# Autodesk Inventor assembly: LowerBody
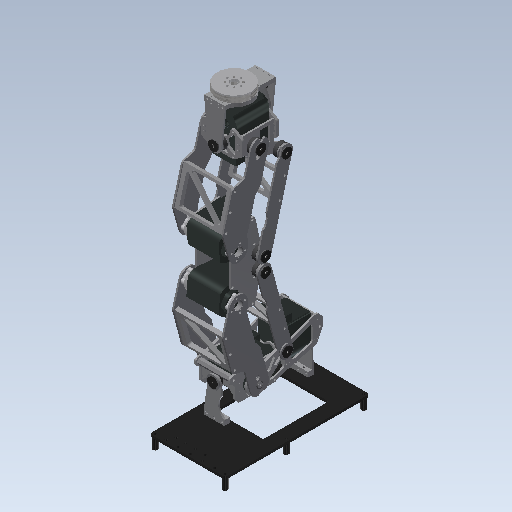
[picture p0: Inventor's stored thumbnail of the model, 512x512]
Saved by Autodesk Inventor 2020.4 (Build 244396000, 396)
## iProperties
Created: 2016-08-23
Part Number: LowerBody
Material: 一般
Document SubType Name: Assembly
Designer: hiro
Mass: 982.556 g
Surface Area: 2608.59 cm^2
Volume: 455.691 cm^3
Density: 2.15619 g/cm^3
Author: hiro
## Documents named in this file (12)
- C:\Users\Masato\Documents\Inventor\CIT Brains_Inventor\OpenPlatform_ver3_0\LowerBody.iam
- C:\Users\Masato\Documents\Inventor\CIT Brains_Inventor\OpenPlatform_ver3_0\下半身\足首\足首_1.iam
- C:\Users\Masato\Documents\Inventor\CIT Brains_Inventor\OpenPlatform_ver3_0\下半身\足首\足首_独立ピッチ_1.iam
- C:\Users\Masato\Documents\Inventor\CIT Brains_Inventor\OpenPlatform_ver3_0\下半身\リンク\LowerFrontLink.iam
- C:\Users\Masato\Documents\Inventor\CIT Brains_Inventor\OpenPlatform_ver3_0\下半身\付け根ロール\付け根ロール_1.iam
- C:\Users\Masato\Documents\Inventor\CIT Brains_Inventor\OpenPlatform_ver3_0\下半身\リンク\LowerBackLink.iam
- C:\Users\Masato\Documents\Inventor\CIT Brains_Inventor\OpenPlatform_ver3_0\下半身\長穴減速\長穴減速_ホーン.iam
- C:\Users\Masato\Documents\Inventor\CIT Brains_Inventor\OpenPlatform_ver3_0\下半身\膝\膝_1.iam
- C:\Users\Masato\Documents\Inventor\CIT Brains_Inventor\OpenPlatform_ver3_0\下半身\付け根\付け根_1.iam
- C:\Users\Masato\Documents\Inventor\CIT Brains_Inventor\OpenPlatform_ver3_0\下半身\リンク\UpperBackLink.iam
- C:\Users\Masato\Documents\Inventor\CIT Brains_Inventor\OpenPlatform_ver3_0\下半身\リンク\UpperFrontLink.iam
- C:\Users\Masato\Documents\Inventor\CIT Brains_Inventor\OpenPlatform_ver3_0\下半身\足裏\foot.iam
## Components (12 placed, 11 different names)
1. 付け根ロール_1:1 [sub-assembly] — メイト:23, フラッシュ:25, フラッシュ:26, 挿入:97, 角度:4, 角度:8, 角度:12, 挿入:123
2. 長穴減速_ホーン:1 [sub-assembly] — 挿入:97, 挿入:109
3. 付け根_1:1 [sub-assembly] — 角度:4, 挿入:109, 挿入:112, 挿入:113, 挿入:123
4. UpperFrontLink:1 [sub-assembly] — 挿入:111, 挿入:112, 角度:12
5. UpperBackLink:1 [sub-assembly] — 挿入:113, 挿入:114
6. 膝_1:1 [sub-assembly] — 挿入:98, 挿入:111, 挿入:114, 挿入:115
7. LowerFrontLink:2 [sub-assembly] — 挿入:98, 角度:11, 挿入:118
8. LowerBackLink:1 [sub-assembly] — 挿入:115, 挿入:120, 挿入:122
9. 足首_1:1 [sub-assembly] — 挿入:117, 挿入:119, 挿入:121
10. 足首_独立ピッチ_1:1 [sub-assembly] — 挿入:118, 挿入:119, 挿入:120
11. 足首_独立ピッチ_1:2 [sub-assembly] — 挿入:121, 挿入:122
12. Foot:1 [sub-assembly] — 角度:8, 挿入:117, 角度:11
## Relationships (22: Insert 15, Angle 4, Flush 2, Mate 1)
- メイト:23 [Mate]: 付け根ロール_1:1
- フラッシュ:25 [Flush]: 付け根ロール_1:1
- フラッシュ:26 [Flush]: 付け根ロール_1:1
- 挿入:97 [Insert]: 付け根ロール_1:1 ↔ 長穴減速_ホーン:1
- 挿入:98 [Insert]: 膝_1:1 ↔ LowerFrontLink:2
- 角度:4 [Angle] (0 deg): 付け根ロール_1:1 ↔ 付け根_1:1
- 挿入:109 [Insert]: 長穴減速_ホーン:1 ↔ 付け根_1:1
- 挿入:111 [Insert]: UpperFrontLink:1 ↔ 膝_1:1
- 挿入:112 [Insert]: 付け根_1:1 ↔ UpperFrontLink:1
- 挿入:113 [Insert]: 付け根_1:1 ↔ UpperBackLink:1
- 挿入:114 [Insert]: UpperBackLink:1 ↔ 膝_1:1
- 挿入:115 [Insert]: 膝_1:1 ↔ LowerBackLink:1
- 角度:8 [Angle] (0 deg): 付け根ロール_1:1 ↔ Foot:1
- 挿入:117 [Insert]: 足首_1:1 ↔ Foot:1
- 角度:11 [Angle] (15 deg): LowerFrontLink:2 ↔ Foot:1
- 角度:12 [Angle] (15 deg): 付け根ロール_1:1 ↔ UpperFrontLink:1
- 挿入:118 [Insert]: LowerFrontLink:2 ↔ 足首_独立ピッチ_1:1
- 挿入:119 [Insert]: 足首_1:1 ↔ 足首_独立ピッチ_1:1
- 挿入:120 [Insert]: LowerBackLink:1 ↔ 足首_独立ピッチ_1:1
- 挿入:121 [Insert]: 足首_1:1 ↔ 足首_独立ピッチ_1:2
- 挿入:122 [Insert]: LowerBackLink:1 ↔ 足首_独立ピッチ_1:2
- 挿入:123 [Insert]: 付け根ロール_1:1 ↔ 付け根_1:1
